# Autodesk Inventor assembly: Assembly2
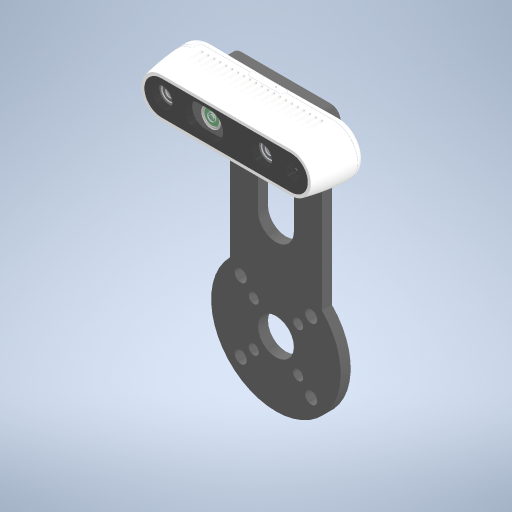
[picture p0: Inventor's stored thumbnail of the model, 512x512]
Saved by Autodesk Inventor 2023 (Build 270158000, 158)
## iProperties
Created: 2022-09-08
Part Number: Assembly2
Document SubType Name: Assembly
Designer: romanp
Author: romanp
## Documents named in this file (3)
- C:\Users\romanp\Desktop\Assembly2.iam
- C:\Users\romanp\Downloads\RealSense_D435i_+_Holder\STEP\Part_Type_2_Black.ipt
- C:\Users\romanp\Downloads\RealSense_D435i_+_Holder\STEP\IntelRealsense_D435.ipt
## Components (2 placed, 2 different names)
1. Part_Type_2_Black:1 — Insert:1, Insert:2
2. IntelRealsense_D435:1 — Insert:1, Insert:2
## Relationships (2: Insert 2)
- Insert:1: Part_Type_2_Black:1 ↔ IntelRealsense_D435:1
- Insert:2: Part_Type_2_Black:1 ↔ IntelRealsense_D435:1
